# Autodesk Inventor assembly: en_son_total_montaj
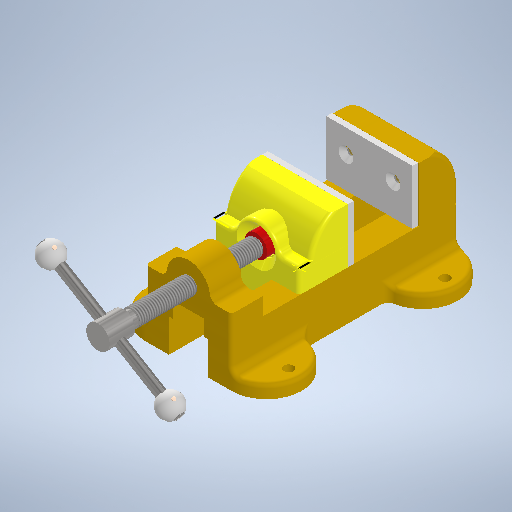
[picture p0: Inventor's stored thumbnail of the model, 512x512]
Saved by Autodesk Inventor 2025.4 (Build 294407000, 407)
## iProperties
Created: 2026-06-22
Part Number: en_son_total_montaj
Document SubType Name: Assembly
Designer: win10
Author: win10
## Documents named in this file (5)
- C:\Users\win10\Desktop\cad-final-projesi\en_son_total_montaj.iam
- C:\Users\win10\Desktop\cad-final-projesi\alt_plaka.ipt
- C:\Users\win10\Desktop\cad-final-projesi\haraketli_palaka.ipt
- C:\Users\win10\Desktop\cad-final-projesi\plaka.ipt
- C:\Users\win10\Desktop\cad-final-projesi\VİDA_MİLİ2.iam
## Components (5 placed, 4 different names)
1. alt_plaka:1 — Mate:1, Mate:2, Mate:3, Mate:4, Mate:5, Mate:10
2. haraketli_palaka:1 — Mate:1, Mate:2, Mate:6, Mate:7, Mate:8, Mate:9
3. plaka:1 — Mate:3, Mate:4, Mate:5
4. plaka:2 — Mate:6, Mate:7, Mate:8
5. VİDA_MİLİ2:1 [sub-assembly] — Mate:9, Mate:10
## Relationships (10: Mate 10)
- Mate:1: alt_plaka:1 ↔ haraketli_palaka:1
- Mate:2: alt_plaka:1 ↔ haraketli_palaka:1
- Mate:3: alt_plaka:1 ↔ plaka:1
- Mate:4: alt_plaka:1 ↔ plaka:1
- Mate:5: alt_plaka:1 ↔ plaka:1
- Mate:6: haraketli_palaka:1 ↔ plaka:2
- Mate:7: haraketli_palaka:1 ↔ plaka:2
- Mate:8: haraketli_palaka:1 ↔ plaka:2
- Mate:9: haraketli_palaka:1 ↔ VİDA_MİLİ2:1
- Mate:10: alt_plaka:1 ↔ VİDA_MİLİ2:1
